# Autodesk Inventor assembly: Complete Device
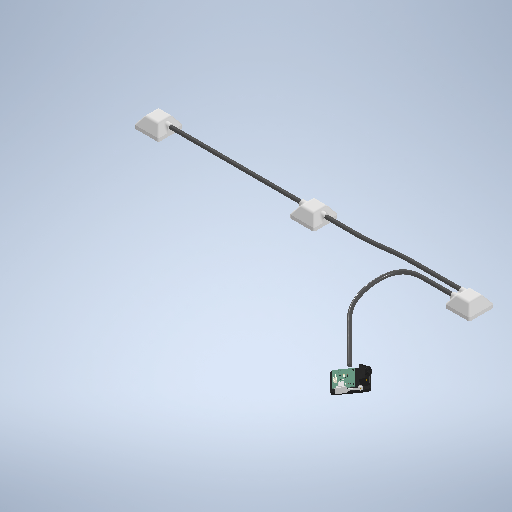
[picture p0: Inventor's stored thumbnail of the model, 512x512]
Saved by Autodesk Inventor 2025.2 (Build 292293000, 293)
## iProperties
Created: 2024-11-20
Part Number: Complete Device
Document SubType Name: Assembly
Designer: tills
Author: tills
## Documents named in this file (8)
- C:\Users\tills\Desktop\Studium\Semester_3\Repositorys\Wearable-Health-Device\Complete Device.iam
- C:\Users\tills\Desktop\Studium\Semester_3\Repositorys\Wearable-Health-Device\Inventor_AKTUELL\ASM IMU mitte.iam
- C:\Users\tills\Desktop\Studium\Semester_3\Repositorys\Wearable-Health-Device\Inventor_AKTUELL\ASM IMU unten.iam
- C:\Users\tills\Desktop\Studium\Semester_3\Repositorys\Wearable-Health-Device\ASM Main.iam
- C:\Users\tills\Desktop\Studium\Semester_3\Repositorys\Wearable-Health-Device\kabel.ipt
- C:\Users\tills\Desktop\Studium\Semester_3\Repositorys\Wearable-Health-Device\Inventor_AKTUELL\ASM IMU oben.iam
- C:\Users\tills\Desktop\Studium\Semester_3\Repositorys\Wearable-Health-Device\kabel2.ipt
- C:\Users\tills\Desktop\Studium\Semester_3\Repositorys\Wearable-Health-Device\Kabel3.ipt
## Components (7 placed, 7 different names)
1. ASM IMU mitte:1 [sub-assembly] — Passend:3, Passend:4, Fluchtend:1, Fluchtend:2, Passend:5, Passend:6, Passend:7, Passend:14, Passend:15, Passend:16, Fluchtend:3
2. ASM IMU unten:1 [sub-assembly] — Passend:1, Passend:2, Fluchtend:3, Winkel:3
3. ASM Main:1 [sub-assembly] — Passend:11, Passend:12, Winkel:2
4. kabel:1 — Passend:1, Passend:2, Passend:3, Passend:4, Winkel:3
5. ASM IMU oben:1 [sub-assembly] — Fluchtend:1, Fluchtend:2, Passend:8, Passend:9, Passend:10, Winkel:1, Passend:13
6. kabel2:1 — Passend:5, Passend:6, Passend:7, Passend:8, Passend:13
7. Kabel3:1 — Passend:9, Passend:10, Winkel:1, Passend:11, Passend:12, Winkel:2
## Relationships (22: Mate 16, Flush 3, Angle 3)
- Passend:1 [Mate]: ASM IMU unten:1 ↔ kabel:1
- Passend:2 [Mate]: ASM IMU unten:1 ↔ kabel:1
- Passend:3 [Mate]: ASM IMU mitte:1 ↔ kabel:1
- Passend:4 [Mate]: ASM IMU mitte:1 ↔ kabel:1
- Fluchtend:1 [Flush]: ASM IMU mitte:1 ↔ ASM IMU oben:1
- Fluchtend:2 [Flush]: ASM IMU mitte:1 ↔ ASM IMU oben:1
- Passend:5 [Mate]: ASM IMU mitte:1 ↔ kabel2:1
- Passend:6 [Mate]: ASM IMU mitte:1 ↔ kabel2:1
- Passend:7 [Mate]: ASM IMU mitte:1 ↔ kabel2:1
- Passend:8 [Mate]: ASM IMU oben:1 ↔ kabel2:1
- Passend:9 [Mate]: ASM IMU oben:1 ↔ Kabel3:1
- Passend:10 [Mate]: ASM IMU oben:1 ↔ Kabel3:1
- Winkel:1 [Angle] (-10 deg): ASM IMU oben:1 ↔ Kabel3:1
- Passend:11 [Mate]: ASM Main:1 ↔ Kabel3:1
- Passend:12 [Mate]: ASM Main:1 ↔ Kabel3:1
- Winkel:2 [Angle] (0 deg): ASM Main:1 ↔ Kabel3:1
- Passend:13 [Mate]: ASM IMU oben:1 ↔ kabel2:1
- Passend:14 [Mate]: ASM IMU mitte:1
- Passend:15 [Mate]: ASM IMU mitte:1
- Passend:16 [Mate]: ASM IMU mitte:1
- Fluchtend:3 [Flush]: ASM IMU mitte:1 ↔ ASM IMU unten:1
- Winkel:3 [Angle] (0 deg): ASM IMU unten:1 ↔ kabel:1
